# Autodesk Inventor assembly: CL-6-F
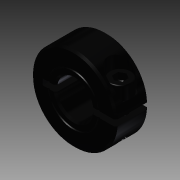
[picture p0: Inventor's stored thumbnail of the model, 180x180]
Saved by Autodesk Inventor 2014 (Build 180170000, 170)
## iProperties
Category: Miscellaneous
Company: Autodesk Inc.
Created: 2013-12-18
Part Number: CL-6-F
Document SubType Name: Assembly
Designer: Autodesk Inc.
Catalog Web Link: http://www.ruland.com/shaft-collar.php?recordID=CL-6-F
Description: 3/8" ID 7/8" OD Clamp Shaft Collar
Vendor: Ruland Manufacturing
Author: Autodesk Inc.
## Documents named in this file (3)
- D:\Data Folder\FIRST 2014\KOP Parts\Miscellaneous\MISC_ShaftCollar_CL-6-F.iam
- D:\Data Folder\FIRST 2014\KOP Parts\Miscellaneous\Parts\ANSI B18.3 - 6-32 UNC - 0.375(31).ipt
- D:\Data Folder\FIRST 2014\KOP Parts\Miscellaneous\Parts\MISC_ShaftCollar_CL-6-F.ipt
## Components (2 placed, 2 different names)
1. MISC_ShaftCollar_CL-6-F:1 — Insert:1
2. Hexagon Socket Head Cap Screw - Inch No. 6 - 32 UNC - 3/8:1 — Insert:1
## Relationships (1: Insert 1)
- Insert:1: MISC_ShaftCollar_CL-6-F:1 ↔ Hexagon Socket Head Cap Screw - Inch No. 6 - 32 UNC - 3/8:1
